# Autodesk Inventor assembly: assembly
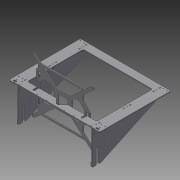
[picture p0: Inventor's stored thumbnail of the model, 180x180]
Saved by Autodesk Inventor 2013 (Build 170138000, 138)
## iProperties
Created: 2013-11-17
Part Number: assembly
Document SubType Name: Assembly
Designer: Masta
Author: Masta
## Documents named in this file (4)
- D:\prusa i3\frame\lasercut_aluminium\assembly.iam
- D:\prusa i3\frame\lasercut_aluminium\caddy.ipt
- D:\prusa i3\frame\lasercut_aluminium\main_frame.ipt
- D:\prusa i3\frame\lasercut_aluminium\side_frame.ipt
## Components (4 placed, 3 different names)
1. main_frame:1 — Mate:1, Flush:3, Mate:2, Mate:3, Mate:4, Flush:4
2. caddy:1 — Mate:4, Flush:4
3. side_frame:1 — Flush:1, Flush:2, Flush:3, Mate:3
4. side_frame:2 — Flush:1, Mate:1, Flush:2, Mate:2
## Relationships (8: Flush 4, Mate 4)
- Flush:1: side_frame:1 ↔ side_frame:2
- Mate:1: main_frame:1 ↔ side_frame:2
- Flush:2: side_frame:1 ↔ side_frame:2
- Flush:3: main_frame:1 ↔ side_frame:1
- Mate:2 (0.25 mm): main_frame:1 ↔ side_frame:2
- Mate:3 (0.25 mm): main_frame:1 ↔ side_frame:1
- Mate:4 (5 mm): main_frame:1 ↔ caddy:1
- Flush:4: main_frame:1 ↔ caddy:1
